# Autodesk Inventor assembly: Aux Cooling Assembly R2
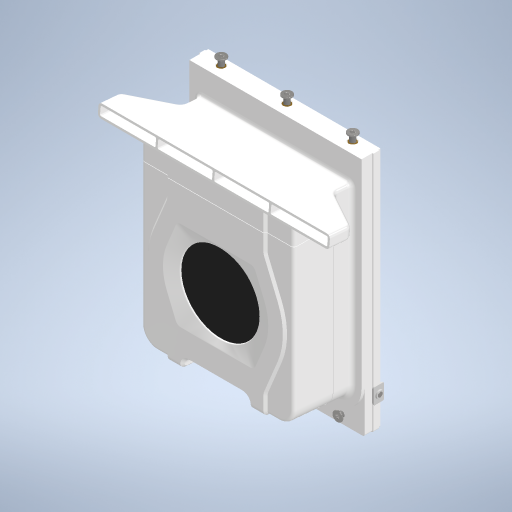
[picture p0: Inventor's stored thumbnail of the model, 512x512]
Saved by Autodesk Inventor 2024 (Build 280153000, 153)
## iProperties
Created: 2024-11-09
Part Number: Aux Cooling Assembly R2
Document SubType Name: Assembly
Designer: Ishaan
Author: Ishaan
## Documents named in this file (12)
- E:\Projects\Axiom--IDEX-3D-Printer\CAD\07 - Auxiliary Cooling\Aux Cooling Assembly R2.iam
- E:\Projects\Axiom--IDEX-3D-Printer\CAD\07 - Auxiliary Cooling\Aux Cooling Case R2.ipt
- E:\Projects\Axiom--IDEX-3D-Printer\CAD\00 - COTS Components\12032 Fan\SanAce_9BFB_120x32_BLW\SanAce_9BFB_120x32_BLW.ipt
- E:\Projects\Axiom--IDEX-3D-Printer\CAD\00 - COTS Components\Hardware\SHCSM4x14.ipt
- E:\Projects\Axiom--IDEX-3D-Printer\CAD\00 - COTS Components\Hardware\M4 LOCKNUT.ipt
- E:\Projects\Axiom--IDEX-3D-Printer\CAD\00 - COTS Components\Hardware\M5 LOCKNUT.ipt
- E:\Projects\Axiom--IDEX-3D-Printer\CAD\00 - COTS Components\HEPA Filter.ipt
- E:\Projects\Axiom--IDEX-3D-Printer\CAD\00 - COTS Components\Hardware\SHCSM5x25.ipt
- E:\Projects\Axiom--IDEX-3D-Printer\CAD\00 - COTS Components\Hardware\Low Profile M5x12.ipt
- E:\Projects\Axiom--IDEX-3D-Printer\CAD\00 - COTS Components\Hardware\SHCSM5x20.ipt
- E:\Projects\Axiom--IDEX-3D-Printer\CAD\00 - COTS Components\Hardware\M5 T SLOT NUT.ipt
- E:\Projects\Axiom--IDEX-3D-Printer\CAD\00 - COTS Components\Hardware\M5 Heat Set Insert.ipt
## Components (29 placed, 11 different names)
1. Aux Cooling Case R2:1 — Insert:1, Insert:2, Insert:3, Insert:4, Insert:5, Insert:6, Insert:15, Insert:16, Insert:17, Angle:6, Angle:7, Angle:8, Mate:1, Mate:2, Mate:3, Insert:18, Insert:19, Insert:20, Insert:21, Insert:22, Insert:23, Insert:24, Insert:25, Angle:9, Insert:26, Angle:10, Insert:27, Insert:28, Insert:29, Insert:30, Insert:31, Insert:32, Insert:33, Insert:34
2. SanAce_9BFB_120x32_BLW:1 — Insert:1, Insert:2, Insert:3, Insert:7, Insert:8, Insert:9
3. SHCSM4x14:1 — Insert:4
4. SHCSM4x14:2 — Insert:5
5. SHCSM4x14:3 — Insert:6
6. M4 LOCKNUT:1 — Insert:7
7. M4 LOCKNUT:2 — Insert:8
8. M4 LOCKNUT:3 — Insert:9
9. M5 LOCKNUT:6 — Insert:15, Angle:6
10. M5 LOCKNUT:7 — Insert:16, Angle:7
11. M5 LOCKNUT:8 — Insert:17, Angle:8
12. HEPA Filter:1 — Mate:1, Mate:2, Mate:3
13. SHCSM5x25:1 — Insert:18
14. SHCSM5x25:2 — Insert:19
15. Low Profile M5x12:1 — Insert:22
16. Low Profile M5x12:2 — Insert:21
17. Low Profile M5x12:3 — Insert:20
18. SHCSM5x20:1 — Insert:23
19. SHCSM5x20:2 — Insert:24
20. M5 T SLOT NUT:1 — Insert:25, Angle:9
21. M5 T SLOT NUT:2 — Insert:26, Angle:10
22. Low Profile M5x12:4 — Insert:32
23. Low Profile M5x12:5 — Insert:33
24. Low Profile M5x12:6 — Insert:34
25. M5 Heat Set Insert:1 — Insert:27
26. M5 Heat Set Insert:2 — Insert:28
27. M5 Heat Set Insert:3 — Insert:29
28. M5 Heat Set Insert:4 — Insert:30
29. M5 Heat Set Insert:5 — Insert:31
## Relationships (37: Insert 29, Angle 5, Mate 3)
- Insert:1: Aux Cooling Case R2:1 ↔ SanAce_9BFB_120x32_BLW:1
- Insert:2: Aux Cooling Case R2:1 ↔ SanAce_9BFB_120x32_BLW:1
- Insert:3: Aux Cooling Case R2:1 ↔ SanAce_9BFB_120x32_BLW:1
- Insert:4: Aux Cooling Case R2:1 ↔ SHCSM4x14:1
- Insert:5: Aux Cooling Case R2:1 ↔ SHCSM4x14:2
- Insert:6: Aux Cooling Case R2:1 ↔ SHCSM4x14:3
- Insert:7: SanAce_9BFB_120x32_BLW:1 ↔ M4 LOCKNUT:1
- Insert:8: SanAce_9BFB_120x32_BLW:1 ↔ M4 LOCKNUT:2
- Insert:9: SanAce_9BFB_120x32_BLW:1 ↔ M4 LOCKNUT:3
- Insert:15: Aux Cooling Case R2:1 ↔ M5 LOCKNUT:6
- Insert:16: Aux Cooling Case R2:1 ↔ M5 LOCKNUT:7
- Insert:17: Aux Cooling Case R2:1 ↔ M5 LOCKNUT:8
- Angle:6 (0 deg): Aux Cooling Case R2:1 ↔ M5 LOCKNUT:6
- Angle:7 (0 deg): Aux Cooling Case R2:1 ↔ M5 LOCKNUT:7
- Angle:8 (0 deg): Aux Cooling Case R2:1 ↔ M5 LOCKNUT:8
- Mate:1 (0.5 mm): Aux Cooling Case R2:1 ↔ HEPA Filter:1
- Mate:2: Aux Cooling Case R2:1 ↔ HEPA Filter:1
- Mate:3 (0.5 mm): Aux Cooling Case R2:1 ↔ HEPA Filter:1
- Insert:18: Aux Cooling Case R2:1 ↔ SHCSM5x25:1
- Insert:19: Aux Cooling Case R2:1 ↔ SHCSM5x25:2
- Insert:20 (3 mm): Aux Cooling Case R2:1 ↔ Low Profile M5x12:3
- Insert:21 (3 mm): Aux Cooling Case R2:1 ↔ Low Profile M5x12:2
- Insert:22 (3 mm): Aux Cooling Case R2:1 ↔ Low Profile M5x12:1
- Insert:23: Aux Cooling Case R2:1 ↔ SHCSM5x20:1
- Insert:24: Aux Cooling Case R2:1 ↔ SHCSM5x20:2
- Insert:25 (2 mm): Aux Cooling Case R2:1 ↔ M5 T SLOT NUT:1
- Angle:9 (0 deg): Aux Cooling Case R2:1 ↔ M5 T SLOT NUT:1
- Insert:26 (2 mm): Aux Cooling Case R2:1 ↔ M5 T SLOT NUT:2
- Angle:10 (0 deg): Aux Cooling Case R2:1 ↔ M5 T SLOT NUT:2
- Insert:27 (0.1 mm): Aux Cooling Case R2:1 ↔ M5 Heat Set Insert:1
- Insert:28 (0.1 mm): Aux Cooling Case R2:1 ↔ M5 Heat Set Insert:2
- Insert:29 (0.1 mm): Aux Cooling Case R2:1 ↔ M5 Heat Set Insert:3
- Insert:30 (0.1 mm): Aux Cooling Case R2:1 ↔ M5 Heat Set Insert:4
- Insert:31 (0.1 mm): Aux Cooling Case R2:1 ↔ M5 Heat Set Insert:5
- Insert:32 (6.35 mm): Aux Cooling Case R2:1 ↔ Low Profile M5x12:4
- Insert:33 (6.35 mm): Aux Cooling Case R2:1 ↔ Low Profile M5x12:5
- Insert:34 (6.35 mm): Aux Cooling Case R2:1 ↔ Low Profile M5x12:6
